# Autodesk Inventor assembly: robot_top
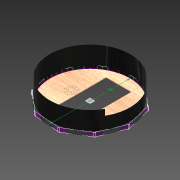
[picture p0: Inventor's stored thumbnail of the model, 180x180]
Saved by Autodesk Inventor 2020 (Build 240168000, 168)
## iProperties
Created: 2022-08-27
Part Number: robot_top
Document SubType Name: Assembly
Designer: Umair
Author: Umair
## Documents named in this file (4)
- C:\Users\pc\Dropbox\Umair\SCHOOL\1 Ma\Masterthesis\CAD\robot_top.iam
- C:\Users\pc\Dropbox\Umair\SCHOOL\1 Ma\Masterthesis\CAD\topplate.ipt
- C:\Users\pc\Dropbox\Umair\SCHOOL\1 Ma\Masterthesis\CAD\Casing_holder.ipt
- C:\Users\pc\Dropbox\Umair\SCHOOL\1 Ma\Masterthesis\CAD\border.ipt
## Components (12 placed, 3 different names)
1. topplate:1 — Mate:1, Mate:2, Mate:4, Mate:6, Mate:22, Flush:9
2. Casing_holder:1 — Mate:4, Mate:5, Mate:9, Mate:20
3. border:1 — Mate:1, Mate:2, Mate:5, Mate:7, Mate:8, Mate:12, Mate:13, Mate:14, Mate:15, Mate:16, Mate:17, Mate:24, Flush:9
4. Casing_holder:2 — Mate:11, Flush:8, Mate:12, Mate:18
5. Casing_holder:3 — Mate:13, Mate:22, Mate:23
6. Casing_holder:4 — Mate:6, Mate:7, Mate:10, Mate:11, Flush:8
7. Casing_holder:6 — Flush:5, Mate:24, Mate:25
8. Casing_holder:7 — Flush:4, Flush:5, Mate:8, Mate:9, Mate:10
9. Casing_holder:8 — Flush:3, Flush:4, Mate:15, Mate:19, Mate:25
10. Casing_holder:9 — Flush:2, Flush:3, Mate:16, Mate:21, Mate:23
11. Casing_holder:10 — Flush:1, Flush:2, Mate:17, Mate:18, Mate:19
12. Casing_holder:11 — Flush:1, Mate:14, Mate:20, Mate:21
## Relationships (31: Mate 24, Flush 7)
- Mate:1: topplate:1 ↔ border:1
- Mate:2: topplate:1 ↔ border:1
- Mate:4: topplate:1 ↔ Casing_holder:1
- Mate:5: Casing_holder:1 ↔ border:1
- Flush:1: Casing_holder:10 ↔ Casing_holder:11
- Flush:2: Casing_holder:9 ↔ Casing_holder:10
- Flush:3: Casing_holder:8 ↔ Casing_holder:9
- Flush:4: Casing_holder:7 ↔ Casing_holder:8
- Flush:5: Casing_holder:6 ↔ Casing_holder:7
- Mate:6: topplate:1 ↔ Casing_holder:4
- Mate:7: border:1 ↔ Casing_holder:4
- Mate:8: border:1 ↔ Casing_holder:7
- Mate:9: Casing_holder:1 ↔ Casing_holder:7
- Mate:10: Casing_holder:4 ↔ Casing_holder:7
- Mate:11: Casing_holder:2 ↔ Casing_holder:4
- Flush:8: Casing_holder:2 ↔ Casing_holder:4
- Mate:12: border:1 ↔ Casing_holder:2
- Mate:13: border:1 ↔ Casing_holder:3
- Mate:14: border:1 ↔ Casing_holder:11
- Mate:15: border:1 ↔ Casing_holder:8
- Mate:16: border:1 ↔ Casing_holder:9
- Mate:17: border:1 ↔ Casing_holder:10
- Mate:18: Casing_holder:2 ↔ Casing_holder:10
- Mate:19: Casing_holder:8 ↔ Casing_holder:10
- Mate:20: Casing_holder:1 ↔ Casing_holder:11
- Mate:21: Casing_holder:9 ↔ Casing_holder:11
- Mate:22: topplate:1 ↔ Casing_holder:3
- Mate:23: Casing_holder:3 ↔ Casing_holder:9
- Mate:24: border:1 ↔ Casing_holder:6
- Mate:25: Casing_holder:6 ↔ Casing_holder:8
- Flush:9: topplate:1 ↔ border:1
